# Autodesk Inventor assembly: ENSAMBLE GENERAL ACH-40L-2020-V
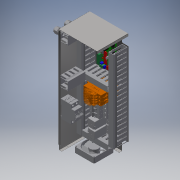
[picture p0: Inventor's stored thumbnail of the model, 180x180]
Saved by Autodesk Inventor 2017 (Build 210142000, 142)
## iProperties
Created: 2020-09-24
Part Number: ENSAMBLE GENERAL ACH-40L-2020-V
Description: STEP AP203
Document SubType Name: Assembly
Designer: USUARIO
Sending System: SolidWorks 2013
Preprocessor: SwSTEP 2.0
Title: ENSAMBLE GENERAL ACH-40L-2020-V.STEP
Revision Number: ANY
## Documents named in this file (51)
- D:\Laboratorio\Autoclave\Autoclave Horizontal\Sin Precamara\2020\Autoclave 40L con Vacio Insulab #0045883XX OP2020292\ENSAMBLE GENERAL ACH-40L-2020-V.iam
- D:\Laboratorio\Autoclave\Autoclave Horizontal\Sin Precamara\2020\Autoclave 40L con Vacio Insulab #0045883XX OP2020292\CUBIERTA FRONTAL ACH-40L-2020-V.ipt
- D:\Laboratorio\Autoclave\Autoclave Horizontal\Sin Precamara\2020\Autoclave 40L con Vacio Insulab #0045883XX OP2020292\BASE MUEBLE ACH-40L-2020-V.ipt
- D:\Laboratorio\Autoclave\Autoclave Horizontal\Sin Precamara\2020\Autoclave 40L con Vacio Insulab #0045883XX OP2020292\MARCO POSTERIOR ACH-40L-2020-V.ipt
- D:\Laboratorio\Autoclave\Autoclave Horizontal\Sin Precamara\2020\Autoclave 40L con Vacio Insulab #0045883XX OP2020292\ENSAMBLE TANQUE ACH-40L-2020-V.iam
- D:\Laboratorio\Autoclave\Autoclave Horizontal\Sin Precamara\2020\Autoclave 40L con Vacio Insulab #0045883XX OP2020292\ENSAMBLE PANEL FRONTAL ACH-40L-2020-V.iam
- D:\Laboratorio\Autoclave\Autoclave Horizontal\Sin Precamara\2020\Autoclave 40L con Vacio Insulab #0045883XX OP2020292\ENSAMBLE PUERTA ACH-40L-2020-V.iam
- D:\Laboratorio\Autoclave\Autoclave Horizontal\Sin Precamara\2020\Autoclave 40L con Vacio Insulab #0045883XX OP2020292\CAJA CONEXIONES ESPINAS ACH-40L-2020-V.ipt
- D:\Laboratorio\Autoclave\Autoclave Horizontal\Sin Precamara\2020\Autoclave 40L con Vacio Insulab #0045883XX OP2020292\PG-13,5.ipt
- D:\Laboratorio\Autoclave\Autoclave Horizontal\Sin Precamara\2020\Autoclave 40L con Vacio Insulab #0045883XX OP2020292\CAJA CONEXIONES ACH-40L-2020-V.ipt
- D:\Laboratorio\Autoclave\Autoclave Horizontal\Sin Precamara\2020\Autoclave 40L con Vacio Insulab #0045883XX OP2020292\REFUERZO INTERIOR ACH-40L-2020-V.ipt
- D:\Laboratorio\Autoclave\Autoclave Horizontal\Sin Precamara\2020\Autoclave 40L con Vacio Insulab #0045883XX OP2020292\VENTILADOR 9X9.ipt
- D:\Laboratorio\Autoclave\Autoclave Horizontal\Sin Precamara\2020\Autoclave 40L con Vacio Insulab #0045883XX OP2020292\ENSAMBLE GENERAL CIERRE JP2019-TTNR.iam
- D:\Laboratorio\Autoclave\Autoclave Horizontal\Sin Precamara\2020\Autoclave 40L con Vacio Insulab #0045883XX OP2020292\PIN CIERRE JP2019-TTNR.ipt
- D:\Laboratorio\Autoclave\Autoclave Horizontal\Sin Precamara\2020\Autoclave 40L con Vacio Insulab #0045883XX OP2020292\PIN BISAGRA JP2019-TTNR.ipt
- D:\Laboratorio\Autoclave\Autoclave Horizontal\Sin Precamara\2020\Autoclave 40L con Vacio Insulab #0045883XX OP2020292\PIVOTE CIERRE JP2019-TTNR.ipt
- D:\Laboratorio\Autoclave\Autoclave Horizontal\Sin Precamara\2020\Autoclave 40L con Vacio Insulab #0045883XX OP2020292\ENSAMBLE TAPA ACH-40L-2020-V.iam
- D:\Laboratorio\Autoclave\Autoclave Horizontal\Sin Precamara\2020\Autoclave 40L con Vacio Insulab #0045883XX OP2020292\ENSAMBLE RESERVORIO ACH-40L-2020-V.iam
- D:\Laboratorio\Autoclave\Autoclave Horizontal\Sin Precamara\2020\Autoclave 40L con Vacio Insulab #0045883XX OP2020292\CONTRATAPA SUPERIOR ACH-40L-2020-V.ipt
- D:\Laboratorio\Autoclave\Autoclave Horizontal\Sin Precamara\2020\Autoclave 40L con Vacio Insulab #0045883XX OP2020292\BANDEJA INTERIOR ACH-40L-2020-V.ipt
- D:\Laboratorio\Autoclave\Autoclave Horizontal\Sin Precamara\2020\Autoclave 40L con Vacio Insulab #0045883XX OP2020292\BOMBA DE VACIO THOMAS 2107CA20.ipt
- D:\Laboratorio\Autoclave\Autoclave Horizontal\Sin Precamara\2020\Autoclave 40L con Vacio Insulab #0045883XX OP2020292\CALDERIN ACH-40L-2020-V.ipt
- D:\Laboratorio\Autoclave\Autoclave Horizontal\Sin Precamara\2020\Autoclave 40L con Vacio Insulab #0045883XX OP2020292\CONTRATAPA INFERIOR ACH-40L-2020-V.ipt
- D:\Laboratorio\Autoclave\Autoclave Horizontal\Sin Precamara\2020\Autoclave 40L con Vacio Insulab #0045883XX OP2020292\CUBIERTA SUPERIOR ACH-40L-2020-V.ipt
- D:\Laboratorio\Autoclave\Autoclave Horizontal\Sin Precamara\2020\Autoclave 40L con Vacio Insulab #0045883XX OP2020292\CUBIERTA LATERAL ACH-40L-2020-V.ipt
- D:\Laboratorio\Autoclave\Autoclave Horizontal\Sin Precamara\2020\Autoclave 40L con Vacio Insulab #0045883XX OP2020292\ENSAMBLE RADIADOR ACH-40L-2020-V.iam
- D:\Laboratorio\Autoclave\Autoclave Horizontal\Sin Precamara\2020\Autoclave 40L con Vacio Insulab #0045883XX OP2020292\CUBIERTA LATERAL DERECHA ACH-40L-2020-V.ipt
- D:\Laboratorio\Autoclave\Autoclave Horizontal\Sin Precamara\2020\Autoclave 40L con Vacio Insulab #0045883XX OP2020292\CUBIERTA POSTERIOR ACH-40L-2020-V.ipt
- D:\Laboratorio\Autoclave\Autoclave Horizontal\Sin Precamara\2020\Autoclave 40L con Vacio Insulab #0045883XX OP2020292\ULKA EX5.ipt
- D:\Laboratorio\Autoclave\Autoclave Horizontal\Sin Precamara\2020\Autoclave 40L con Vacio Insulab #0045883XX OP2020292\DANFOSS EV215B.ipt
- D:\Laboratorio\Autoclave\Autoclave Horizontal\Sin Precamara\2020\Autoclave 40L con Vacio Insulab #0045883XX OP2020292\SOPORTE BOMBA AGUA ACH-40L-2020-V.ipt
- D:\Laboratorio\Autoclave\Autoclave Horizontal\Sin Precamara\2020\Autoclave 40L con Vacio Insulab #0045883XX OP2020292\SOPORTE VALVULAS ACH-40L-2020-V.ipt
- D:\Laboratorio\Autoclave\Autoclave Horizontal\Sin Precamara\2020\Autoclave 40L con Vacio Insulab #0045883XX OP2020292\PATA 5-16.ipt
- D:\Laboratorio\Autoclave\Autoclave Horizontal\Sin Precamara\2020\Autoclave 40L con Vacio Insulab #0045883XX OP2020292\VALVULA DE BOLA GENEBRE MH 3097-02 CW617N.ipt
- D:\Laboratorio\Autoclave\Autoclave Horizontal\Sin Precamara\2020\Autoclave 40L con Vacio Insulab #0045883XX OP2020292\ESPINAS DE PESCADO ACV-ACH.ipt
- D:\Laboratorio\Autoclave\Autoclave Horizontal\Sin Precamara\2020\Autoclave 40L con Vacio Insulab #0045883XX OP2020292\DERIVACION TANQUE ACH-40L-2020-V.ipt
- D:\Laboratorio\Autoclave\Autoclave Horizontal\Sin Precamara\2020\Autoclave 40L con Vacio Insulab #0045883XX OP2020292\TEE VALVULAS ACH-40L-2020-V.ipt
- D:\Laboratorio\Autoclave\Autoclave Horizontal\Sin Precamara\2020\Autoclave 40L con Vacio Insulab #0045883XX OP2020292\RESISTENCIA INTERIOR ACH-40L-2020-V.ipt
- D:\Laboratorio\Autoclave\Autoclave Horizontal\Sin Precamara\2020\Autoclave 40L con Vacio Insulab #0045883XX OP2020292\RESISTENCIA SECADO ACH-40L-2020-V.ipt
- D:\Laboratorio\Autoclave\Autoclave Horizontal\Sin Precamara\2020\Autoclave 40L con Vacio Insulab #0045883XX OP2020292\DEFLECTOR ACH-40L-2020-V.ipt
- D:\Laboratorio\Autoclave\Autoclave Horizontal\Sin Precamara\2020\Autoclave 40L con Vacio Insulab #0045883XX OP2020292\ACOPLE DEFLECTOR ACH-40L-2020-V.ipt
- D:\Laboratorio\Autoclave\Autoclave Horizontal\Sin Precamara\2020\Autoclave 40L con Vacio Insulab #0045883XX OP2020292\Schematic\Nextion Control SM\NextionControlV3.iam
- C:\Modelos 3D y DXF\Rele Relpol 2C\R15 2P.ipt
- C:\Modelos 3D y DXF\Rele Relpol 2C\PZ8.ipt
- C:\Modelos 3D y DXF\Ex9C 25-38-NOARK.stp\Ex9C 25-38-NOARK.ipt
- C:\Modelos 3D y DXF\B1A-NOARK.stp\75856.ipt
- C:\Users\USUARIO\Documents\Inventor\Canaleta 30x60 450mm.iam
- C:\Users\USUARIO\Documents\Inventor\Canaleta 30x60 120mm.iam
- C:\Users\USUARIO\Documents\Inventor\Canaleta 30x60 380mm.iam
- C:\Users\USUARIO\Documents\Inventor\Canaleta 40x40 80mm.iam
- C:\Modelos 3D y DXF\Prensacables\User Library-BUD CABLE GLAND.ipt
## Components (68 placed, 61 different names)
1. CUBIERTA FRONTAL ACH-40L-2020-V_1
2. BASE MUEBLE ACH-40L-2020-V_2
3. MARCO POSTERIOR ACH-40L-2020-V_3
4. ENSAMBLE PANEL FRONTAL ACH-40L-2020-V_5 [sub-assembly]
5. ENSAMBLE PUERTA ACH-40L-2020-V_6 [sub-assembly] — Mate:5, Flush:1, Flush:2
6. CAJA CONEXIONES ESPINAS ACH-40L-2020-V_7
7. PG-13,5_8
8. CAJA CONEXIONES ACH-40L-2020-V_9 — Mate:1, Mate:2, Mate:6, Angle:1, Mate:9, Angle:2, Angle:3, Mate:12, Mate:23, Angle:4, Mate:24, Angle:5, Mate:25, Mate:26, Mate:27, Mate:28, Mate:29, Mate:30, Mate:31, Mate:32, Mate:33, Mate:34, Mate:35, Mate:37, Mate:38, Mate:39, Mate:40, Mate:41, Mate:43, Mate:44, Mate:45, Angle:6
9. REFUERZO INTERIOR ACH-40L-2020-V_10
10. REFUERZO INTERIOR ACH-40L-2020-V_11
11. VENTILADOR 9X9_12
12. ENSAMBLE GENERAL CIERRE JP2019-TTNR_13 [sub-assembly]
13. PIN CIERRE JP2019-TTNR_14
14. PIN BISAGRA JP2019-TTNR_15 — Insert:1
15. PIN BISAGRA JP2019-TTNR_16
16. PIVOTE CIERRE JP2019-TTNR_17
17. ENSAMBLE TAPA ACH-40L-2020-V_18 [sub-assembly] — Insert:1, Insert:2, Insert:3
18. ENSAMBLE RESERVORIO ACH-40L-2020-V_19 [sub-assembly]
19. CONTRATAPA SUPERIOR ACH-40L-2020-V_20 — Insert:2, Mate:5, Flush:1, Flush:2
20. BANDEJA INTERIOR ACH-40L-2020-V_21
21. BOMBA DE VACIO THOMAS 2107CA20_22
22. CALDERIN ACH-40L-2020-V_23
23. CONTRATAPA INFERIOR ACH-40L-2020-V_24 — Insert:3
24. CUBIERTA SUPERIOR ACH-40L-2020-V_25
25. CUBIERTA LATERAL ACH-40L-2020-V_26
26. ENSAMBLE RADIADOR ACH-40L-2020-V_27 [sub-assembly]
27. CUBIERTA LATERAL DERECHA ACH-40L-2020-V_28
28. CUBIERTA POSTERIOR ACH-40L-2020-V_29
29. ULKA EX5_30
30. DANFOSS EV215B_31
31. SOPORTE BOMBA AGUA ACH-40L-2020-V_32
32. SOPORTE VALVULAS ACH-40L-2020-V_33
33. DANFOSS EV215B_34
34. DANFOSS EV215B_35
35. DANFOSS EV215B_36
36. DANFOSS EV215B_37
37. DANFOSS EV215B_38
38. PATA 5-16_39
39. PATA 5-16_40
40. PATA 5-16_41
41. PATA 5-16_42
42. PG-13,5_43
43. VALVULA DE BOLA GENEBRE MH 3097-02 CW617N_44
44. ESPINAS DE PESCADO ACV-ACH_45
45. DERIVACION TANQUE ACH-40L-2020-V_46
46. TEE VALVULAS ACH-40L-2020-V_47
47. RESISTENCIA INTERIOR ACH-40L-2020-V_48
48. RESISTENCIA SECADO ACH-40L-2020-V_49
49. DEFLECTOR ACH-40L-2020-V_50
50. ACOPLE DEFLECTOR ACH-40L-2020-V_51
51. NextionControlV3:1 [sub-assembly] — Mate:1, Mate:2, Mate:42
52. R15 2P:1 — Mate:7, Mate:8
53. PZ8:1 — Mate:6, Angle:1, Mate:7, Mate:8
54. Ex9C 25-38-NOARK:1 — Mate:9, Angle:2
55. R15 2P:2
56. PZ8:2 — Angle:3, Mate:12
57. 75856:1 — Mate:23, Angle:4
58. 75856:2 — Mate:24, Angle:5
59. Canaleta 30x60 450mm:1 [sub-assembly] — Mate:25, Mate:26, Mate:27, Mate:36
60. Canaleta 30x60 120mm:1 [sub-assembly] — Mate:28, Mate:42
61. Canaleta 30x60 380mm:1 [sub-assembly] — Mate:29, Mate:30, Mate:31
62. Canaleta 40x40 80mm:1 [sub-assembly] — Mate:32, Mate:33, Mate:34
63. Canaleta 30x60 120mm:2 [sub-assembly] — Mate:35, Mate:36, Mate:37
64. User Library-BUD CABLE GLAND:1 — Mate:38, Mate:39, Tangent:1
65. ENSAMBLE TANQUE ACH-40L-2020-V:1 [sub-assembly] — Mate:40
66. User Library-BUD CABLE GLAND:2 — Mate:41, Tangent:1
67. Canaleta 40x40 80mm:2 [sub-assembly] — Mate:43, Mate:44
68. 75856:3 — Mate:45, Angle:6
## Relationships (45: Mate 33, Angle 6, Insert 3, Flush 2, Tangent 1)
- Mate:1 (10 mm): CAJA CONEXIONES ACH-40L-2020-V_9 ↔ NextionControlV3:1
- Mate:2 (10 mm): CAJA CONEXIONES ACH-40L-2020-V_9 ↔ NextionControlV3:1
- Insert:1: PIN BISAGRA JP2019-TTNR_15 ↔ ENSAMBLE TAPA ACH-40L-2020-V_18
- Insert:2: ENSAMBLE TAPA ACH-40L-2020-V_18 ↔ CONTRATAPA SUPERIOR ACH-40L-2020-V_20
- Insert:3: ENSAMBLE TAPA ACH-40L-2020-V_18 ↔ CONTRATAPA INFERIOR ACH-40L-2020-V_24
- Mate:5: ENSAMBLE PUERTA ACH-40L-2020-V_6 ↔ CONTRATAPA SUPERIOR ACH-40L-2020-V_20
- Flush:1 (-5 mm): ENSAMBLE PUERTA ACH-40L-2020-V_6 ↔ CONTRATAPA SUPERIOR ACH-40L-2020-V_20
- Flush:2 (-5 mm): ENSAMBLE PUERTA ACH-40L-2020-V_6 ↔ CONTRATAPA SUPERIOR ACH-40L-2020-V_20
- Mate:6: CAJA CONEXIONES ACH-40L-2020-V_9 ↔ PZ8:1
- Angle:1 (90.4127 deg): CAJA CONEXIONES ACH-40L-2020-V_9 ↔ PZ8:1
- Mate:7: R15 2P:1 ↔ PZ8:1
- Mate:8: R15 2P:1 ↔ PZ8:1
- Mate:9 (-4 mm): CAJA CONEXIONES ACH-40L-2020-V_9 ↔ Ex9C 25-38-NOARK:1
- Angle:2 (0 deg): CAJA CONEXIONES ACH-40L-2020-V_9 ↔ Ex9C 25-38-NOARK:1
- [Mate]: R15 2P:2 ↔ PZ8:2
- [Mate]: R15 2P:2 ↔ PZ8:2
- Angle:3 (0 deg): CAJA CONEXIONES ACH-40L-2020-V_9 ↔ PZ8:2
- Mate:12: CAJA CONEXIONES ACH-40L-2020-V_9 ↔ PZ8:2
- Mate:23: CAJA CONEXIONES ACH-40L-2020-V_9 ↔ 75856:1
- Angle:4 (0 deg): CAJA CONEXIONES ACH-40L-2020-V_9 ↔ 75856:1
- Mate:24: CAJA CONEXIONES ACH-40L-2020-V_9 ↔ 75856:2
- Angle:5 (0 deg): CAJA CONEXIONES ACH-40L-2020-V_9 ↔ 75856:2
- Mate:25: CAJA CONEXIONES ACH-40L-2020-V_9 ↔ Canaleta 30x60 450mm:1
- Mate:26 (4 mm): CAJA CONEXIONES ACH-40L-2020-V_9 ↔ Canaleta 30x60 450mm:1
- Mate:27 (5 mm): CAJA CONEXIONES ACH-40L-2020-V_9 ↔ Canaleta 30x60 450mm:1
- Mate:28: CAJA CONEXIONES ACH-40L-2020-V_9 ↔ Canaleta 30x60 120mm:1
- Mate:29: CAJA CONEXIONES ACH-40L-2020-V_9 ↔ Canaleta 30x60 380mm:1
- Mate:30 (-28 mm): CAJA CONEXIONES ACH-40L-2020-V_9 ↔ Canaleta 30x60 380mm:1
- Mate:31 (5 mm): CAJA CONEXIONES ACH-40L-2020-V_9 ↔ Canaleta 30x60 380mm:1
- Mate:32: CAJA CONEXIONES ACH-40L-2020-V_9 ↔ Canaleta 40x40 80mm:1
- Mate:33: CAJA CONEXIONES ACH-40L-2020-V_9 ↔ Canaleta 40x40 80mm:1
- Mate:34 (5 mm): CAJA CONEXIONES ACH-40L-2020-V_9 ↔ Canaleta 40x40 80mm:1
- Mate:35: CAJA CONEXIONES ACH-40L-2020-V_9 ↔ Canaleta 30x60 120mm:2
- Mate:36: Canaleta 30x60 450mm:1 ↔ Canaleta 30x60 120mm:2
- Mate:37: CAJA CONEXIONES ACH-40L-2020-V_9 ↔ Canaleta 30x60 120mm:2
- Mate:38: CAJA CONEXIONES ACH-40L-2020-V_9 ↔ User Library-BUD CABLE GLAND:1
- Mate:39 (-25 mm): CAJA CONEXIONES ACH-40L-2020-V_9 ↔ User Library-BUD CABLE GLAND:1
- Mate:40: CAJA CONEXIONES ACH-40L-2020-V_9 ↔ ENSAMBLE TANQUE ACH-40L-2020-V:1
- Mate:41: CAJA CONEXIONES ACH-40L-2020-V_9 ↔ User Library-BUD CABLE GLAND:2
- Tangent:1 (20 mm): User Library-BUD CABLE GLAND:1 ↔ User Library-BUD CABLE GLAND:2
- Mate:42 (18 mm): NextionControlV3:1 ↔ Canaleta 30x60 120mm:1
- Mate:43: CAJA CONEXIONES ACH-40L-2020-V_9 ↔ Canaleta 40x40 80mm:2
- Mate:44: CAJA CONEXIONES ACH-40L-2020-V_9 ↔ Canaleta 40x40 80mm:2
- Mate:45: CAJA CONEXIONES ACH-40L-2020-V_9 ↔ 75856:3
- Angle:6 (0 deg): CAJA CONEXIONES ACH-40L-2020-V_9 ↔ 75856:3
## Named parameters: d35_d29 = 0 mm, d36_d30 = 0 mm
